# Autodesk Inventor assembly: 正四方轴套
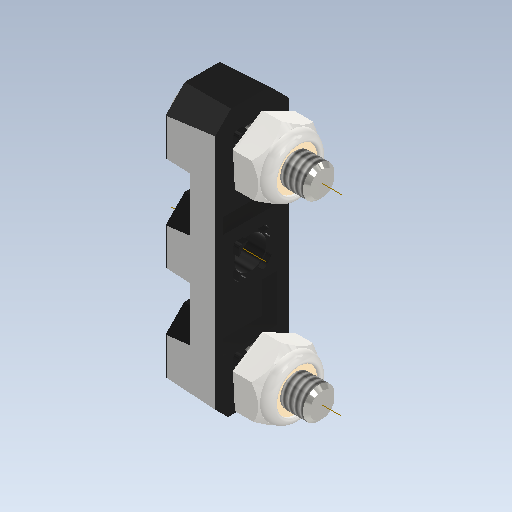
[picture p0: Inventor's stored thumbnail of the model, 512x512]
Saved by Autodesk Inventor 2020 (Build 240168000, 168)
## iProperties
Created: 2019-05-29
Part Number: 正四方轴套
Document SubType Name: Assembly
Designer: aresp
Author: aresp
## Documents named in this file (3)
- D:\Backup\Documents\Vault\ncrCadLib\轴相关\细轴配套\正四方轴套.iam
- D:\Backup\Documents\Vault\ncrCadLib\轴相关\细轴配套\零件\细轴四方轴承.ipt
- D:\Backup\Documents\Vault\ncrCadLib\轴相关\粗轴配套\零件\四号螺丝+防滑.iam
## Components (3 placed, 2 different names)
1. 细轴四方轴承:1 — 配合:1, 配合:2, 配合:3
2. 四号螺丝+防滑:1 [sub-assembly] — 表面齐平:1, 配合:3
3. 四号螺丝+防滑:2 [sub-assembly] — 表面齐平:1, 配合:1, 配合:2
## Relationships (4: Mate 3, Flush 1)
- 表面齐平:1 [Flush]: 四号螺丝+防滑:1 ↔ 四号螺丝+防滑:2
- 配合:1 [Mate]: 细轴四方轴承:1 ↔ 四号螺丝+防滑:2
- 配合:2 [Mate]: 细轴四方轴承:1 ↔ 四号螺丝+防滑:2
- 配合:3 [Mate]: 细轴四方轴承:1 ↔ 四号螺丝+防滑:1
